# Autodesk Inventor assembly: Switch_Micro-L
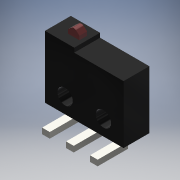
[picture p0: Inventor's stored thumbnail of the model, 180x180]
Saved by Autodesk Inventor 2017 (Build 210142000, 142)
## iProperties
Created: 2013-07-18
Part Number: Switch_Micro-L
Document SubType Name: Assembly
Designer: Bradley
Sending System: SolidWorks 2002025
Preprocessor: SwSTEP 2.0
## Documents named in this file (3)
- C:\Users\Bradley\Documents\CougsInSpace\Resources\ComponentModels\Electronics\Switch_Micro-L.iam
- C:\Users\Bradley\Documents\CougsInSpace\Resources\ComponentModels\Electronics\Components\Switch_Micro-L\D2MQ_1_TL_ACTUATOR.ipt
- C:\Users\Bradley\Documents\CougsInSpace\Resources\ComponentModels\Electronics\Components\Switch_Micro-L\D2MQ_1_TL_BASE.ipt
## Components (2 placed, 2 different names)
1. D2MQ_1_TL_ACTUATOR_1 — Flush:1, Flush:2, Mate:1
2. D2MQ_1_TL_BASE_2 — Flush:1, Flush:2, Mate:1
## Relationships (3: Flush 2, Mate 1)
- Flush:1 (-0.95 mm): D2MQ_1_TL_ACTUATOR_1 ↔ D2MQ_1_TL_BASE_2
- Flush:2 (-1.45 mm): D2MQ_1_TL_ACTUATOR_1 ↔ D2MQ_1_TL_BASE_2
- Mate:1 (-5.7 mm): D2MQ_1_TL_ACTUATOR_1 ↔ D2MQ_1_TL_BASE_2
